# Autodesk Inventor assembly: SHOT_0_000_PivotAssembly
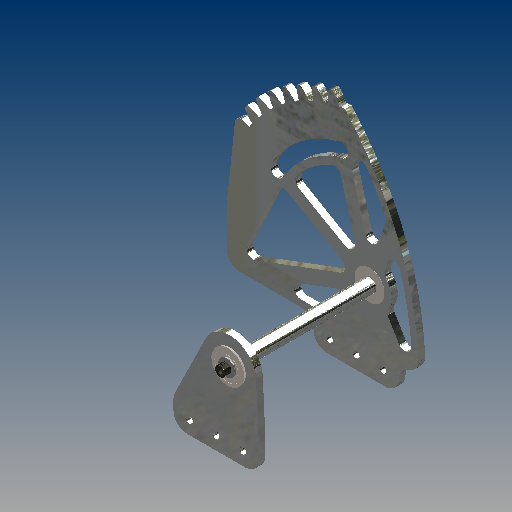
[picture p0: Inventor's stored thumbnail of the model, 512x512]
Saved by Autodesk Inventor 2024.3 (Build 283343000, 343)
## iProperties
Created: 2024-08-07
Part Number: SHOT_0_000_PivotAssembly
Document SubType Name: Assembly
Designer: Bryan
Mass: 708.017 g
Surface Area: 1048.32 cm^2
Volume: 246.247 cm^3
Density: 2.87523 g/cm^3
Author: Bryan
## Documents named in this file (13)
- C:\Users\Kenji\Documents\GitHub\1622-2024-Summer-CAD-A-Thon\Shooter\SHOT_0_000_PivotAssembly.iam
- C:\Users\Kenji\Documents\GitHub\1622-2024-Summer-CAD-A-Thon\Shooter\SHOT_0_001_PivotGear.ipt
- C:\Users\Kenji\Documents\GitHub\1622-2024-Summer-CAD-A-Thon\Shooter\SHOT_0_002_PivotPlate.ipt
- C:\Users\Kenji\Documents\GitHub\1622-2024-Summer-CAD-A-Thon\COTS Library\Motion\Bearings\COTS_WCP-0781_0.5ODCircularFlangedBearing.ipt
- C:\Users\Kenji\Documents\GitHub\1622-2024-Summer-CAD-A-Thon\Shooter\SHOT_0_003_PivotShaft.ipt
- C:\Users\Kenji\Documents\GitHub\1622-2024-Summer-CAD-A-Thon\COTS Library\Fasteners\Bolts\Socket-Head\0.25-20\COTS_91251A540_Black-Oxide Alloy Steel Socket Head Screw.ipt
- C:\Users\Kenji\Documents\GitHub\1622-2024-Summer-CAD-A-Thon\COTS Library\Fasteners\Washers\COTS_90107A029_316 Stainless Steel Washer.ipt
- C:\Users\bobsb\OneDrive\Documents\GitHub\1622-2024-Summer-CAD-A-Thon\Shooter\SHOT_0_000_PivotAssembly\AIP\FEA\es9fun6yo.fins
- C:\Users\bobsb\OneDrive\Documents\GitHub\1622-2024-Summer-CAD-A-Thon\Shooter\SHOT_0_000_PivotAssembly\AIP\FEA\es9fun6yo.fsat
- C:\Users\bobsb\OneDrive\Documents\GitHub\1622-2024-Summer-CAD-A-Thon\Shooter\SHOT_0_000_PivotAssembly\AIP\FEA\es9fun6yo.ftes
- C:\Users\bobsb\OneDrive\Documents\GitHub\1622-2024-Summer-CAD-A-Thon\Shooter\SHOT_0_000_PivotAssembly\AIP\FEA\es9fun6yo.fwiz
- C:\Users\bobsb\OneDrive\Documents\GitHub\1622-2024-Summer-CAD-A-Thon\Shooter\SHOT_0_000_PivotAssembly\AIP\FEA\es9fun728.fmsh
- C:\Users\Kenji\Documents\GitHub\1622-2024-Summer-CAD-A-Thon\Shooter\SHOT_0_000_PivotAssembly\AIP\FEA\es9fun729.fres
## Components (9 placed, 6 different names)
1. SHOT_0_001_PivotGear:1 — Mate:1, Mate:3, Mate:4, Mate:7, Mate:8
2. SHOT_0_002_PivotPlate:1 — Mate:1, Mate:3, Mate:4, Mate:5, Mate:6
3. COTS_WCP-0781_0.5ODCircularFlangedBearing:1 — Mate:5, Mate:6
4. COTS_WCP-0781_0.5ODCircularFlangedBearing:2 — Mate:7, Mate:8, Mate:9, Flush:1
5. SHOT_0_003_PivotShaft:1 — Mate:9, Flush:1, Mate:10, Mate:11, Mate:12, Mate:13, Mate:15, Mate:16
6. COTS_91251A540_Black-Oxide Alloy Steel Socket Head Screw:1 — Mate:10, Mate:17
7. COTS_91251A540_Black-Oxide Alloy Steel Socket Head Screw:2 — Mate:11, Mate:14
8. COTS_90107A029_316 Stainless Steel Washer:1 — Mate:12, Mate:13, Mate:14
9. COTS_90107A029_316 Stainless Steel Washer:2 — Mate:15, Mate:16, Mate:17
## Relationships (17: Mate 16, Flush 1)
- Mate:1: SHOT_0_001_PivotGear:1 ↔ SHOT_0_002_PivotPlate:1
- Mate:3 (127 mm): SHOT_0_001_PivotGear:1 ↔ SHOT_0_002_PivotPlate:1
- Mate:4: SHOT_0_001_PivotGear:1 ↔ SHOT_0_002_PivotPlate:1
- Mate:5: SHOT_0_002_PivotPlate:1 ↔ COTS_WCP-0781_0.5ODCircularFlangedBearing:1
- Mate:6: SHOT_0_002_PivotPlate:1 ↔ COTS_WCP-0781_0.5ODCircularFlangedBearing:1
- Mate:7: SHOT_0_001_PivotGear:1 ↔ COTS_WCP-0781_0.5ODCircularFlangedBearing:2
- Mate:8: SHOT_0_001_PivotGear:1 ↔ COTS_WCP-0781_0.5ODCircularFlangedBearing:2
- Mate:9: COTS_WCP-0781_0.5ODCircularFlangedBearing:2 ↔ SHOT_0_003_PivotShaft:1
- Flush:1: COTS_WCP-0781_0.5ODCircularFlangedBearing:2 ↔ SHOT_0_003_PivotShaft:1
- Mate:10: SHOT_0_003_PivotShaft:1 ↔ COTS_91251A540_Black-Oxide Alloy Steel Socket Head Screw:1
- Mate:11: SHOT_0_003_PivotShaft:1 ↔ COTS_91251A540_Black-Oxide Alloy Steel Socket Head Screw:2
- Mate:12: SHOT_0_003_PivotShaft:1 ↔ COTS_90107A029_316 Stainless Steel Washer:1
- Mate:13: SHOT_0_003_PivotShaft:1 ↔ COTS_90107A029_316 Stainless Steel Washer:1
- Mate:14: COTS_91251A540_Black-Oxide Alloy Steel Socket Head Screw:2 ↔ COTS_90107A029_316 Stainless Steel Washer:1
- Mate:15: SHOT_0_003_PivotShaft:1 ↔ COTS_90107A029_316 Stainless Steel Washer:2
- Mate:16: SHOT_0_003_PivotShaft:1 ↔ COTS_90107A029_316 Stainless Steel Washer:2
- Mate:17: COTS_91251A540_Black-Oxide Alloy Steel Socket Head Screw:1 ↔ COTS_90107A029_316 Stainless Steel Washer:2
## Named parameters: sa_0 = 13344.7
note: some values were not read from the file. Shown as the stored number, unit unknown: "sa_0".
